# Autodesk Inventor assembly: ASY PNS 1650 filter-distribution-system 1000
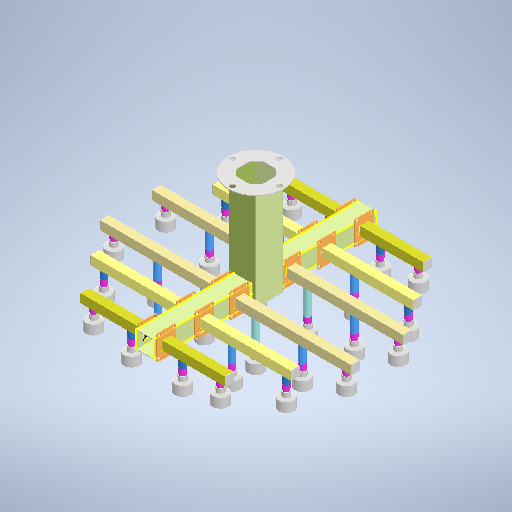
[picture p0: Inventor's stored thumbnail of the model, 512x512]
Saved by Autodesk Inventor 2025 (Build 290162010, 162A)
## iProperties
Created: 2025-06-24
Part Number: ASY PNS 1650 filter-distribution-system 1000
Document SubType Name: Assembly
Designer: admin
Author: user
## Documents named in this file (9)
- C:\Users\pokla\Documents\Inventor\TZS-Tazovskiy\Filter D940\FDS 940\ASY PNS 1650 filter-distribution-system 1000.iam
- C:\Users\pokla\Documents\Inventor\TZS-Tazovskiy\Filter D940\FDS 940\TZS 169859 DIM filter-distribution-system 940.ipt
- C:\Users\pokla\Documents\Inventor\TZS-Tazovskiy\Filter D940\FDS 940\TZS 1651 FDS MAIN  FLANGE.ipt
- C:\Users\pokla\Documents\Inventor\TZS-Tazovskiy\Filter D940\FDS 940\TZS 1652 FDS Central tube wall.ipt
- C:\Users\pokla\Documents\Inventor\TZS-Tazovskiy\Filter D940\FDS 940\TZS 1653 FDS 940 Diameter beam.ipt
- C:\Users\pokla\Documents\Inventor\TZS-Tazovskiy\Filter D940\FDS 940\ASY TZS FDS way1_940.iam
- C:\Users\pokla\Documents\Inventor\TZS-Tazovskiy\Filter D940\FDS 940\ASY TZS 1662 FDS way 2.iam
- C:\Users\pokla\Documents\Inventor\TZS-Tazovskiy\Filter D940\FDS 940\ASY TZS FDS way3_940.iam
- C:\Users\pokla\Documents\Inventor\TZS-Tazovskiy\Filter D940\FDS 940\TZS 1665 FDS 940 CUP 1.ipt
## Components (19 placed, 9 different names)
1. PNS 169859 DIM filter-distribution-system 1000.ipt:1 — Mate:5, Mate:4
2. PNS 1651 FDS MAIN  FLANGE.ipt:1 — Flush:1, Flush:2, Mate:1
3. PNS 1652 FDS Central tube wall.ipt:1 — Flush:1, Flush:4, Flush:3, Mate:6, Rigid:1, Rigid:2
4. PNS 1652 FDS Central tube wall.ipt:2 — Flush:2, Mate:1, Rigid:1, Rigid:3
5. PNS 1653 FDS 1000 Diameter beam.ipt:1 — Rigid:2, Rigid:4, Rigid:5, Rigid:9, Rigid:14, Rigid:15, Rigid:35
6. PNS 1653 FDS 1000 Diameter beam.ipt:2 — Rigid:3, Rigid:11, Rigid:13, Rigid:12, Rigid:16, Rigid:17, Rigid:34
7. ASY PNS FDS way1_1600.iam:1 [sub-assembly] — Rigid:4
8. ASY PNS 1662 FDS way 2.iam:1 [sub-assembly] — Rigid:5
9. ASY PNS FDS way3_1600.iam:1 [sub-assembly] — Rigid:35
10. ASY PNS FDS way1_1600.iam:2 [sub-assembly] — Rigid:9
11. ASY PNS FDS way1_1600.iam:3 [sub-assembly] — Rigid:11
12. ASY PNS 1662 FDS way 2.iam:2 [sub-assembly] — Rigid:14
13. ASY PNS 1662 FDS way 2.iam:3 [sub-assembly] — Rigid:13
14. ASY PNS 1662 FDS way 2.iam:4 [sub-assembly] — Rigid:12
15. ASY PNS FDS way3_1600.iam:2 [sub-assembly] — Rigid:15
16. ASY PNS FDS way3_1600.iam:3 [sub-assembly] — Rigid:16
17. ASY PNS FDS way3_1600.iam:4 [sub-assembly] — Rigid:17
18. PNS 1665 FDS 1000 CUP 1.ipt:1 — Flush:4, Flush:3, Mate:6
19. ASY PNS FDS way1_1600:4 [sub-assembly] — Rigid:34
## Relationships (23: WeldJoint 15, Mate 4, Flush 4)
- Mate:5: PNS 169859 DIM filter-distribution-system 1000.ipt:1
- Mate:4: PNS 169859 DIM filter-distribution-system 1000.ipt:1
- Flush:1: PNS 1651 FDS MAIN  FLANGE.ipt:1 ↔ PNS 1652 FDS Central tube wall.ipt:1
- Flush:2: PNS 1651 FDS MAIN  FLANGE.ipt:1 ↔ PNS 1652 FDS Central tube wall.ipt:2
- Mate:1: PNS 1651 FDS MAIN  FLANGE.ipt:1 ↔ PNS 1652 FDS Central tube wall.ipt:2
- Flush:4: PNS 1652 FDS Central tube wall.ipt:1 ↔ PNS 1665 FDS 1000 CUP 1.ipt:1
- Flush:3: PNS 1652 FDS Central tube wall.ipt:1 ↔ PNS 1665 FDS 1000 CUP 1.ipt:1
- Mate:6: PNS 1652 FDS Central tube wall.ipt:1 ↔ PNS 1665 FDS 1000 CUP 1.ipt:1
- Rigid:1 [WeldJoint]: PNS 1652 FDS Central tube wall.ipt:1 ↔ PNS 1652 FDS Central tube wall.ipt:2
- Rigid:2 [WeldJoint]: PNS 1652 FDS Central tube wall.ipt:1 ↔ PNS 1653 FDS 1000 Diameter beam.ipt:1
- Rigid:3 [WeldJoint]: PNS 1652 FDS Central tube wall.ipt:2 ↔ PNS 1653 FDS 1000 Diameter beam.ipt:2
- Rigid:4 [WeldJoint] (-2 mm): PNS 1653 FDS 1000 Diameter beam.ipt:1 ↔ ASY PNS FDS way1_1600.iam:1
- Rigid:5 [WeldJoint] (-2 mm): PNS 1653 FDS 1000 Diameter beam.ipt:1 ↔ ASY PNS 1662 FDS way 2.iam:1
- Rigid:9 [WeldJoint]: PNS 1653 FDS 1000 Diameter beam.ipt:1 ↔ ASY PNS FDS way1_1600.iam:2
- Rigid:11 [WeldJoint]: PNS 1653 FDS 1000 Diameter beam.ipt:2 ↔ ASY PNS FDS way1_1600.iam:3
- Rigid:14 [WeldJoint]: PNS 1653 FDS 1000 Diameter beam.ipt:1 ↔ ASY PNS 1662 FDS way 2.iam:2
- Rigid:13 [WeldJoint]: PNS 1653 FDS 1000 Diameter beam.ipt:2 ↔ ASY PNS 1662 FDS way 2.iam:3
- Rigid:12 [WeldJoint]: PNS 1653 FDS 1000 Diameter beam.ipt:2 ↔ ASY PNS 1662 FDS way 2.iam:4
- Rigid:15 [WeldJoint]: PNS 1653 FDS 1000 Diameter beam.ipt:1 ↔ ASY PNS FDS way3_1600.iam:2
- Rigid:16 [WeldJoint]: PNS 1653 FDS 1000 Diameter beam.ipt:2 ↔ ASY PNS FDS way3_1600.iam:3
- Rigid:17 [WeldJoint]: PNS 1653 FDS 1000 Diameter beam.ipt:2 ↔ ASY PNS FDS way3_1600.iam:4
- Rigid:34 [WeldJoint]: PNS 1653 FDS 1000 Diameter beam.ipt:2 ↔ ASY PNS FDS way1_1600:4
- Rigid:35 [WeldJoint]: PNS 1653 FDS 1000 Diameter beam.ipt:1 ↔ ASY PNS FDS way3_1600.iam:1
